# Autodesk Inventor assembly: EnsamblajeSalon
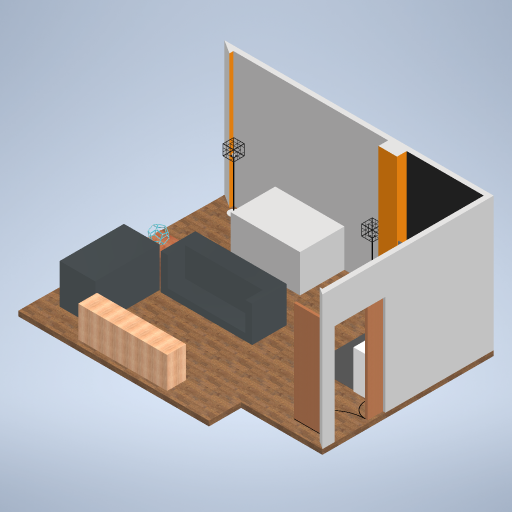
[picture p0: Inventor's stored thumbnail of the model, 512x512]
Saved by Autodesk Inventor 2024 (Build 280153000, 153)
## iProperties
Created: 2024-04-05
Part Number: EnsamblajeSalon
Document SubType Name: Assembly
Designer: sergi
Author: sergi
## Documents named in this file (20)
- C:\Users\sergi\OneDrive\Escritorio\Projects\07. Home\Living room\Inventor\EnsamblajeSalon.iam
- C:\Users\sergi\OneDrive\Escritorio\Projects\07. Home\Living room\Inventor\Paredes.ipt
- C:\Users\sergi\OneDrive\Escritorio\Projects\07. Home\Living room\Inventor\Ventana.ipt
- C:\Users\sergi\OneDrive\Escritorio\Projects\07. Home\Living room\Inventor\Suelo.ipt
- C:\Users\sergi\OneDrive\Escritorio\Projects\07. Home\Living room\Inventor\Puerta.ipt
- C:\Users\sergi\OneDrive\Escritorio\Projects\07. Home\Living room\Inventor\PuertaPequeña.ipt
- C:\Users\sergi\OneDrive\Escritorio\Projects\07. Home\Desk\Inventor\DeskV2\Escritorio2.iam
- C:\Users\sergi\OneDrive\Escritorio\Projects\07. Home\Living room\Inventor\tinker.ipt
- C:\Users\sergi\OneDrive\Escritorio\Projects\07. Home\Living room\Inventor\Pantalla.ipt
- C:\Users\sergi\OneDrive\Escritorio\Projects\07. Home\Living room\Inventor\Mueble Tele.ipt
- C:\Users\sergi\OneDrive\Escritorio\Projects\07. Home\Living room\Inventor\Sofa Pequeño.ipt
- C:\Users\sergi\OneDrive\Escritorio\Projects\07. Home\Living room\Inventor\Mesa Comedor.ipt
- C:\Users\sergi\OneDrive\Escritorio\Projects\07. Home\Living room\Inventor\Ensamblaje Lampara.iam
- C:\Users\sergi\OneDrive\Escritorio\Projects\07. Home\Kumiko lamp\Inventor\sofa.ipt
- C:\Users\sergi\OneDrive\Escritorio\Projects\07. Home\Living room\Inventor\Mesa Pequeña.ipt
- C:\Users\sergi\OneDrive\Escritorio\Projects\07. Home\Living room\Inventor\Mueble Acuario.ipt
- C:\Users\sergi\OneDrive\Escritorio\Projects\07. Home\Living room\Inventor\Acuario.ipt
- C:\Users\sergi\OneDrive\Escritorio\Projects\07. Home\Living room\Inventor\Alfombras.ipt
- C:\Users\sergi\OneDrive\Escritorio\Projects\07. Home\Living room\Inventor\Mesita.ipt
- C:\Users\sergi\OneDrive\Escritorio\Projects\01. Infinity dodecahedron\Inventor\EnsamblajeDodecaedro_V3.iam
## Components (21 placed, 19 different names)
1. Paredes:1 — Nivelación:1, Nivelación:2, Nivelación:3, Ángulo:1, Coincidencia:2, Coincidencia:3, Coincidencia:4, Coincidencia:7, Coincidencia:8, Coincidencia:11, Coincidencia:12, Coincidencia:13, Nivelación:21, Coincidencia:21, Coincidencia:23, Coincidencia:24
2. Ventana:1 — Nivelación:1
3. Suelo:1 — Nivelación:2, Nivelación:3, Nivelación:6, Nivelación:7, Coincidencia:1, Coincidencia:5, Nivelación:9, Nivelación:10, Nivelación:13, Nivelación:14, Nivelación:15, Nivelación:16, Coincidencia:18, Coincidencia:19, Coincidencia:20, Nivelación:17, Nivelación:18, Nivelación:19, Nivelación:20, Nivelación:24, Nivelación:25, Nivelación:26, Coincidencia:24
4. Puerta:1 — Ángulo:1, Coincidencia:1, Coincidencia:2
5. PuertaPequeña:1 — Nivelación:6, Nivelación:7
6. Escritorio2:1 [sub-assembly] — Coincidencia:3, Coincidencia:4, Coincidencia:5, Coincidencia:6, Coincidencia:9, Coincidencia:10, Coincidencia:22
7. tinker:1 — Coincidencia:6, Coincidencia:7, Coincidencia:8
8. Pantalla:1 — Coincidencia:10, Nivelación:8
9. Pantalla:2 — Coincidencia:9, Nivelación:8
10. Mueble Tele:1 — Nivelación:9, Nivelación:10, Coincidencia:11, Coincidencia:12
11. Sofa Pequeño:1 — Nivelación:13, Nivelación:14
12. Mesa Comedor:1 — Nivelación:15, Nivelación:16, Coincidencia:13
13. Ensamblaje Lampara:1 [sub-assembly] — Coincidencia:18
14. Ensamblaje Lampara:2 [sub-assembly] — Coincidencia:19
15. sofa:1 — Coincidencia:20
16. Mesa Pequeña:1 — Nivelación:17, Nivelación:18
17. Mueble Acuario:1 — Nivelación:19, Nivelación:20, Nivelación:21, Coincidencia:21, Nivelación:22, Nivelación:23
18. Acuario:1 — Nivelación:22, Nivelación:23
19. Alfombras:1 — Nivelación:24, Nivelación:25, Coincidencia:22, Coincidencia:23
20. Mesita:1 — Nivelación:26
21. EnsamblajeDodecaedro_V3:1 [sub-assembly]
## Relationships (43: Flush 22, Mate 20, Angle 1)
- Nivelación:1 [Flush]: Paredes:1 ↔ Ventana:1
- Nivelación:2 [Flush]: Paredes:1 ↔ Suelo:1
- Nivelación:3 [Flush]: Paredes:1 ↔ Suelo:1
- Nivelación:6 [Flush]: Suelo:1 ↔ PuertaPequeña:1
- Nivelación:7 [Flush]: Suelo:1 ↔ PuertaPequeña:1
- Ángulo:1 [Angle] (-90 deg): Paredes:1 ↔ Puerta:1
- Coincidencia:1 [Mate]: Suelo:1 ↔ Puerta:1
- Coincidencia:2 [Mate]: Paredes:1 ↔ Puerta:1
- Coincidencia:3 [Mate]: Paredes:1 ↔ Escritorio2:1
- Coincidencia:4 [Mate]: Paredes:1 ↔ Escritorio2:1
- Coincidencia:5 [Mate]: Suelo:1 ↔ Escritorio2:1
- Coincidencia:6 [Mate] (10 mm): Escritorio2:1 ↔ tinker:1
- Coincidencia:7 [Mate] (50 mm): Paredes:1 ↔ tinker:1
- Coincidencia:8 [Mate] (100 mm): Paredes:1 ↔ tinker:1
- Coincidencia:9 [Mate]: Escritorio2:1 ↔ Pantalla:2
- Coincidencia:10 [Mate]: Escritorio2:1 ↔ Pantalla:1
- Nivelación:8 [Flush]: Pantalla:1 ↔ Pantalla:2
- Nivelación:9 [Flush]: Suelo:1 ↔ Mueble Tele:1
- Nivelación:10 [Flush]: Suelo:1 ↔ Mueble Tele:1
- Coincidencia:11 [Mate]: Paredes:1 ↔ Mueble Tele:1
- Coincidencia:12 [Mate] (480 mm): Paredes:1 ↔ Mueble Tele:1
- Nivelación:13 [Flush]: Suelo:1 ↔ Sofa Pequeño:1
- Nivelación:14 [Flush]: Suelo:1 ↔ Sofa Pequeño:1
- Nivelación:15 [Flush]: Suelo:1 ↔ Mesa Comedor:1
- Nivelación:16 [Flush]: Suelo:1 ↔ Mesa Comedor:1
- Coincidencia:13 [Mate]: Paredes:1 ↔ Mesa Comedor:1
- Coincidencia:18 [Mate]: Suelo:1 ↔ Ensamblaje Lampara:1
- Coincidencia:19 [Mate]: Suelo:1 ↔ Ensamblaje Lampara:2
- Coincidencia:20 [Mate]: Suelo:1 ↔ sofa:1
- Nivelación:17 [Flush]: Suelo:1 ↔ Mesa Pequeña:1
- Nivelación:18 [Flush]: Suelo:1 ↔ Mesa Pequeña:1
- Nivelación:19 [Flush]: Suelo:1 ↔ Mueble Acuario:1
- Nivelación:20 [Flush]: Suelo:1 ↔ Mueble Acuario:1
- Nivelación:21 [Flush]: Paredes:1 ↔ Mueble Acuario:1
- Coincidencia:21 [Mate]: Paredes:1 ↔ Mueble Acuario:1
- Nivelación:22 [Flush]: Mueble Acuario:1 ↔ Acuario:1
- Nivelación:23 [Flush]: Mueble Acuario:1 ↔ Acuario:1
- Nivelación:24 [Flush]: Suelo:1 ↔ Alfombras:1
- Nivelación:25 [Flush]: Suelo:1 ↔ Alfombras:1
- Coincidencia:22 [Mate]: Escritorio2:1 ↔ Alfombras:1
- Coincidencia:23 [Mate] (100 mm): Paredes:1 ↔ Alfombras:1
- Nivelación:26 [Flush]: Suelo:1 ↔ Mesita:1
- Coincidencia:24 [Mate]: Paredes:1 ↔ Suelo:1
